# Autodesk Inventor assembly: AssemblyFull
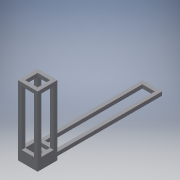
[picture p0: Inventor's stored thumbnail of the model, 180x180]
Saved by Autodesk Inventor 2017 (Build 210142000, 142)
## iProperties
Created: 2019-07-06
Part Number: AssemblyFull
Document SubType Name: Assembly
Designer: Ole Simmering
Author: Ole Simmering
## Documents named in this file (5)
- C:\Users\Ole Simmering\Documents\GitHub\3D_modeling\Guillotine\AssemblyFull.iam
- C:\Users\Ole Simmering\Documents\GitHub\3D_modeling\Guillotine\Assembly.iam
- C:\Users\Ole Simmering\Documents\GitHub\3D_modeling\Guillotine\AssemblyBench.iam
- C:\Users\Ole Simmering\Documents\GitHub\3D_modeling\Guillotine\4ix4ix19i.ipt
- C:\Users\Ole Simmering\Documents\GitHub\3D_modeling\Guillotine\4ix4ix6i.ipt
## Components (5 placed, 4 different names)
1. Assembly:1 [sub-assembly] — Mate:1, Flush:1, Flush:2, Mate:2, Mate:3, Flush:3, Mate:4, Flush:4, Mate:5
2. AssemblyBench:1 [sub-assembly] — Mate:1, Flush:1, Flush:2
3. 4ix4ix19i:1 — Mate:4, Flush:4, Mate:5, Mate:6, Flush:5, Flush:6
4. 4ix4ix19i:2 — Mate:2, Mate:3, Flush:3
5. 4ix4ix6i:1 — Mate:6, Flush:5, Flush:6
## Relationships (12: Mate 6, Flush 6)
- Mate:1: Assembly:1 ↔ AssemblyBench:1
- Flush:1: Assembly:1 ↔ AssemblyBench:1
- Flush:2: Assembly:1 ↔ AssemblyBench:1
- Mate:2: Assembly:1 ↔ 4ix4ix19i:2
- Mate:3: Assembly:1 ↔ 4ix4ix19i:2
- Flush:3: Assembly:1 ↔ 4ix4ix19i:2
- Mate:4: Assembly:1 ↔ 4ix4ix19i:1
- Flush:4: Assembly:1 ↔ 4ix4ix19i:1
- Mate:5: Assembly:1 ↔ 4ix4ix19i:1
- Mate:6: 4ix4ix19i:1 ↔ 4ix4ix6i:1
- Flush:5: 4ix4ix19i:1 ↔ 4ix4ix6i:1
- Flush:6: 4ix4ix19i:1 ↔ 4ix4ix6i:1
